# Autodesk Inventor assembly: V0.2R1 Tulip Mod master v35
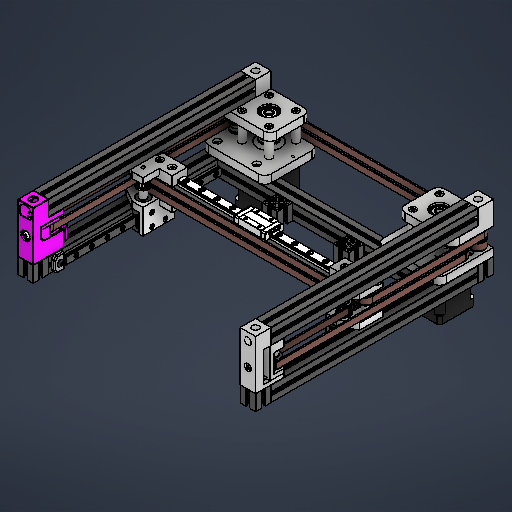
[picture p0: Inventor's stored thumbnail of the model, 512x512]
Saved by Autodesk Inventor 2026 (Build 300175050, 175E)
## iProperties
Created: 2025-05-23
Part Number: V0.2R1 Tulip Mod master v35
Document SubType Name: Assembly
Designer: Joshua Eah
Sending System: Autodesk Translation Framework v13.20.0.188
Preprocessor: ST-DEVELOPER v20
Title: V0.2R1 Tulip Mod master v35.step
## Documents named in this file (7)
- C:\Users\Joshua Eah\Documents\GitHub\Voron-0\CAD\Tulip - Machined Parts\Tulip Mod Master\Master Assembly.iam
- C:\Users\Joshua Eah\Documents\GitHub\Voron-0\CAD\Tulip - Machined Parts\Tulip Mod Master\Frame.iam
- C:\Users\Joshua Eah\Documents\GitHub\Voron-0\CAD\Tulip - Machined Parts\Tulip Mod Master\X Axis (1).iam
- C:\Users\Joshua Eah\Documents\GitHub\Voron-0\CAD\Tulip - Machined Parts\AB Drives\A Drive\A_Drive.iam
- C:\Users\Joshua Eah\Documents\GitHub\Voron-0\CAD\Tulip - Machined Parts\AB Drives\B Drive\B_Drive.iam
- C:\Users\Joshua Eah\Documents\GitHub\Voron-0\CAD\Tulip - Machined Parts\V0.2R1 Tulip Mod Live Idlers v4\Tension_Idler_B_Live.iam
- C:\Users\Joshua Eah\Documents\GitHub\Voron-0\CAD\Tulip - Machined Parts\Idlers\Idler Assembly.iam
## Components (6 placed, 6 different names)
1. Frame:1 [sub-assembly] — Insert:1, Angle:1, Insert:4, Insert:5
2. X Axis:1 [sub-assembly]
3. A_Drive:1 [sub-assembly]
4. B_Drive:1 [sub-assembly] — Insert:1, Angle:1
5. Tension_Idler_B_Live:1 [sub-assembly]
6. Idler Assembly:1 [sub-assembly] — Insert:4, Insert:5
## Relationships (6: Insert 5, Angle 1)
- Insert:1: Frame:1 ↔ B_Drive:1
- Angle:1 (0 deg): Frame:1 ↔ B_Drive:1
- [Insert]: Frame:1 ↔ X Axis:1
- [Insert]: Frame:1 ↔ X Axis:1
- Insert:4: Frame:1 ↔ Idler Assembly:1
- Insert:5: Frame:1 ↔ Idler Assembly:1
